# Autodesk Inventor assembly: 0002_Part_Khop_tay_1
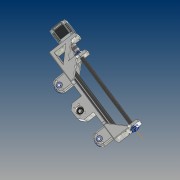
[picture p0: Inventor's stored thumbnail of the model, 180x180]
Saved by Autodesk Inventor 2021 (Build 250183000, 183)
## iProperties
Created: 2024-04-01
Part Number: 0002_Part_Khop_tay_1
Document SubType Name: Assembly
Designer: Admin
Mass: 1057.6 g
Surface Area: 2364.91 cm^2
Volume: 894.304 cm^3
Density: 1.18259 g/cm^3
Author: Admin
## Documents named in this file (9)
- C:\Users\Admin\Desktop\DO_AN_TOT_NGHIEP_2024\Mechanical\Design_in_3D\Version_2\0002_Part_Khop_tay_1.iam
- C:\Users\Admin\Desktop\DO_AN_TOT_NGHIEP_2024\Mechanical\Design_in_3D\Version_1\15_Khop_trung_gian.ipt
- C:\Users\Admin\Desktop\DO_AN_TOT_NGHIEP_2024\Mechanical\Design_in_3D\Library\hgr-20-1.snapshot.3\Modify_KyAnh\Thanh_truot_20x200.ipt
- C:\Users\Admin\Desktop\DO_AN_TOT_NGHIEP_2024\Mechanical\Design_in_3D\Library\Vit_me_300x12.ipt
- C:\Users\Admin\Desktop\Do_an\Ver_3\Thu_vien\KFL_08_3\KFL08 - Mancal Flange oval Ø8.ipt
- C:\Users\Admin\Desktop\DO_AN_TOT_NGHIEP_2024\Mechanical\Design_in_3D\Library\stepper-motor-flexible-coupling-6-35-x-8-mm-1.snapshot.2\Stepper Motor Flexible Coupling 6,35 x 8 mm.iam
- C:\Users\Admin\Desktop\DO_AN_TOT_NGHIEP_2024\Mechanical\Design_in_3D\Library\nema-23hs5628-1.snapshot.4\NEMA_235628-6.35_s_TOP.iam
- C:\Users\Admin\Desktop\DO_AN_TOT_NGHIEP_2024\Mechanical\Design_in_3D\Library\Truc_vit_1405\Dai_oc_truc_vit.ipt
- C:\Users\Admin\Desktop\DO_AN_TOT_NGHIEP_2024\Mechanical\Design_in_3D\Library\lmef10uu-linearbearing-1.snapshot.1\LM10UU Ball Bearing.ipt
## Components (10 placed, 8 different names)
1. 15_Khop_trung_gian:1 — Mate:41, Angle:2, Mate:47, Mate:48, Mate:50, Mate:51, Mate:52, Mate:54, Angle:4, Mate:55, Angle:5, Mate:56, Mate:57, Mate:58, Insert:8, Insert:9, Mate:59, Mate:60
2. Thanh_truot_20x200:1 — Mate:41, Angle:2, Mate:47, Mate:58
3. Vit_me_300x12:1 — Insert:5, Insert:6
4. KFL08 - Mancal Flange oval Ø8:1 — Insert:5, Mate:51
5. KFL08 - Mancal Flange oval Ø8:2 — Insert:6, Insert:7, Mate:48, Mate:50, Mate:57
6. Stepper Motor Flexible Coupling 6,35 x 8 mm:1 [sub-assembly] — Insert:7
7. NEMA_235628-6.35_s_TOP:1 [sub-assembly] — Mate:52, Mate:54, Angle:4
8. Dai_oc_truc_vit:1 — Mate:55, Angle:5, Mate:56
9. LM10UU Ball Bearing:1 — Insert:8, Mate:59
10. LM10UU Ball Bearing:2 — Insert:9, Mate:60
## Relationships (21: Mate 13, Insert 5, Angle 3)
- Mate:41: 15_Khop_trung_gian:1 ↔ Thanh_truot_20x200:1
- Angle:2 (0 deg): 15_Khop_trung_gian:1 ↔ Thanh_truot_20x200:1
- Insert:5: Vit_me_300x12:1 ↔ KFL08 - Mancal Flange oval Ø8:1
- Insert:6: Vit_me_300x12:1 ↔ KFL08 - Mancal Flange oval Ø8:2
- Insert:7 (2 mm): KFL08 - Mancal Flange oval Ø8:2 ↔ Stepper Motor Flexible Coupling 6,35 x 8 mm:1
- Mate:47: 15_Khop_trung_gian:1 ↔ Thanh_truot_20x200:1
- Mate:48: 15_Khop_trung_gian:1 ↔ KFL08 - Mancal Flange oval Ø8:2
- Mate:50: 15_Khop_trung_gian:1 ↔ KFL08 - Mancal Flange oval Ø8:2
- Mate:51: 15_Khop_trung_gian:1 ↔ KFL08 - Mancal Flange oval Ø8:1
- Mate:52: 15_Khop_trung_gian:1 ↔ NEMA_235628-6.35_s_TOP:1
- Mate:54: 15_Khop_trung_gian:1 ↔ NEMA_235628-6.35_s_TOP:1
- Angle:4 (0 deg): 15_Khop_trung_gian:1 ↔ NEMA_235628-6.35_s_TOP:1
- Mate:55: 15_Khop_trung_gian:1 ↔ Dai_oc_truc_vit:1
- Angle:5 (0 deg): 15_Khop_trung_gian:1 ↔ Dai_oc_truc_vit:1
- Mate:56: 15_Khop_trung_gian:1 ↔ Dai_oc_truc_vit:1
- Mate:57: 15_Khop_trung_gian:1 ↔ KFL08 - Mancal Flange oval Ø8:2
- Mate:58: 15_Khop_trung_gian:1 ↔ Thanh_truot_20x200:1
- Insert:8: 15_Khop_trung_gian:1 ↔ LM10UU Ball Bearing:1
- Insert:9: 15_Khop_trung_gian:1 ↔ LM10UU Ball Bearing:2
- Mate:59: 15_Khop_trung_gian:1 ↔ LM10UU Ball Bearing:1
- Mate:60: 15_Khop_trung_gian:1 ↔ LM10UU Ball Bearing:2
